# Autodesk Inventor assembly: AMR_assembly
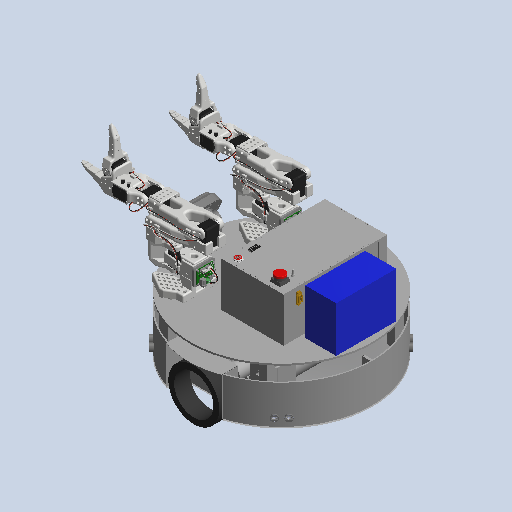
[picture p0: Inventor's stored thumbnail of the model, 512x512]
Saved by Autodesk Inventor 2026 (Build 300175050, 175E)
## iProperties
Part Number: AMR_assembly
Document SubType Name: Assembly
Designer: Kartik
Mass: 9467.85 g
Surface Area: 27408.7 cm^2
Volume: 7326.52 cm^3
Density: 1.29227 g/cm^3
Author: Kartik
## Documents named in this file (23)
- D:\Kartik\Projects\AMR\CAD\1 Assembly\AMR_assembly.iam
- D:\Kartik\Projects\AMR\CAD\3 Parts\AMR_base.ipt
- D:\Kartik\Projects\AMR\CAD\3 Parts\Wheel_Cover.ipt
- D:\Kartik\Projects\AMR\CAD\3 Parts\Wheel_rubber.ipt
- D:\Kartik\Projects\AMR\CAD\3 Parts\Motor.ipt
- D:\Kartik\Projects\AMR\CAD\3 Parts\Motor_mount.ipt
- D:\Kartik\Projects\AMR\CAD\3 Parts\Encoder.ipt
- D:\Kartik\Projects\AMR\CAD\2 Sub-assembly\PCB enclosure.iam
- D:\Kartik\Projects\AMR\CAD\6 Exports\STEP\SO101\SO101 Assembly\SO101 Assembly\SO101 Assembly.iam
- D:\Kartik\Projects\AMR\CAD\3 Parts\Pulley.ipt
- D:\Kartik\Projects\AMR\CAD\3 Parts\Frame_member.ipt
- D:\Kartik\Projects\AMR\CAD\3 Parts\LIdar_p2.ipt
- D:\Kartik\Projects\AMR\CAD\3 Parts\LIdar_p1.ipt
- D:\Kartik\Projects\AMR\CAD\3 Parts\layer2.ipt
- D:\Kartik\Projects\AMR\CAD\3 Parts\Battery.ipt
- D:\Kartik\Projects\AMR\CAD\4 Boughtouts\intel-realsense-depth-camera-d455\INTEL REALSENSE  DEPTH CAMERA D455\INTEL REALSENSE  DEPTH CAMERA D455\INTEL REALSENSE  DEPTH CAMERA D455\INTEL REALSENSE  DEPTH CAMERA D.ipt
- D:\Kartik\Projects\AMR\CAD\4 Boughtouts\intel-realsense-d455-mount-1\Assem1\Assem1\Assem1.ipt
- D:\Kartik\Projects\AMR\CAD\4 Boughtouts\hc-sr04-ultrasonic-sensor-12\Ultrasonic sensor\Ultrasonic sensor\Ultrasonic sensor.ipt
- D:\Kartik\Projects\AMR\CAD\3 Parts\Bottom_Enclosure_1.ipt
- D:\Kartik\Projects\AMR\CAD\3 Parts\Bottom_Enclosure_2.ipt
- D:\Kartik\Projects\AMR\CAD\2 Sub-assembly\PCB enclosure_v2.iam
- D:\Kartik\Projects\AMR\CAD\4 Boughtouts\emergency-stop-switch-1\Emergency stop switch\Emergency stop switch\Emergency stop switch.ipt
- D:\Kartik\Projects\AMR\CAD\4 Boughtouts\mini-toggle-switches-1\6mm SPDT Mini Toggle Switch\6mm SPDT Mini Toggle Switch\6mm SPDT Mini Toggle Switch.ipt
## Components (39 placed, 22 different names)
1. AMR_base:1 — Mate:1, Mate:2, Mate:3, Mate:4, Flush:1, Mate:6, Mate:8, Mate:25, Mate:27, Mate:28, Mate:29, Mate:30, Mate:31, Mate:32, Mate:33, Mate:34, Mate:39, Mate:55, Mate:56, Mate:57, Mate:58, Mate:59, Mate:60, Mate:61, Mate:62
2. Wheel_Cover:1 — Mate:1, Mate:2, Mate:3, Flush:2, Mate:10, Mate:23
3. Wheel_Cover:2 — Mate:4, Flush:1, Flush:2, Mate:9, Mate:24
4. Motor:1 — Flush:5, Mate:7, Flush:6, Mate:18, Mate:26
5. Motor:2 — Flush:3, Mate:5, Flush:4, Mate:16, Mate:25, Mate:26
6. Motor_mount:1 — Flush:5, Mate:7, Flush:6, Mate:8, Mate:17, Mate:24
7. Motor_mount:2 — Flush:3, Mate:5, Flush:4, Mate:6, Mate:15, Mate:23
8. Encoder:1 — Mate:12, Mate:19, Mate:20
9. Encoder:2 — Mate:13, Mate:21, Mate:22
10. Wheel_rubber:2 — Mate:10, Mate:11, Mate:12
11. Wheel_rubber:3 — Mate:9, Mate:11, Mate:13
12. PCB enclosure:1 [sub-assembly] — Mate:40
13. SO101 Assembly:1 [sub-assembly] — Mate:43, Flush:16, Mate:45, Flush:17
14. SO101 Assembly:2 [sub-assembly] — Mate:44, Flush:16, Mate:45, Flush:17
15. Pulley:1 — Mate:15, Mate:16
16. Pulley:2 — Mate:17, Mate:18
17. Pulley:3 — Mate:19, Mate:20
18. Pulley:4 — Mate:21, Mate:22
19. Frame_member:1 — Mate:27, Mate:28, Flush:14, Flush:15
20. Frame_member:2 — Mate:29, Mate:34, Flush:13
21. Frame_member:3 — Mate:30, Mate:33, Flush:13, Flush:14
22. Frame_member:4 — Mate:31, Mate:32, Flush:15
23. LIdar_p2:1 — Mate:36, Mate:37
24. LIdar_p1:1 — Mate:36, Mate:37, Mate:38
25. layer2:1 — Mate:39, Mate:40, Mate:43, Mate:44, Mate:49, Mate:38, Mate:75, Mate:76
26. Battery:1 — Mate:76, Mate:77
27. INTEL REALSENSE  DEPTH CAMERA D:1 — Mate:50, Mate:51, Mate:52
28. Assem1:1 — Mate:49, Mate:50, Mate:51, Mate:52
29. Ultrasonic sensor:1 — Mate:73, Mate:74
30. Ultrasonic sensor:2 — Mate:68, Mate:69
31. Ultrasonic sensor:3 — Mate:66, Mate:67
32. Ultrasonic sensor:4 — Mate:71, Mate:72
33. Bottom_Enclosure_1:1 — Mate:55, Mate:56, Mate:68, Mate:69
34. Bottom_Enclosure_1:2 — Mate:57, Mate:58, Mate:66, Mate:67, Mate:70
35. Bottom_Enclosure_2:1 — Mate:59, Mate:60, Mate:73, Mate:74
36. Bottom_Enclosure_2:2 — Mate:61, Mate:62, Mate:70, Mate:71, Mate:72
37. PCB enclosure_v2:1 [sub-assembly] — Mate:75, Mate:77, Mate:78, Mate:79
38. Emergency stop switch:1 — Mate:78
39. 6mm SPDT Mini Toggle Switch:1 — Mate:79
## Relationships (78: Mate 67, Flush 11)
- Mate:1: AMR_base:1 ↔ Wheel_Cover:1
- Mate:2: AMR_base:1 ↔ Wheel_Cover:1
- Mate:3: AMR_base:1 ↔ Wheel_Cover:1
- Mate:4: AMR_base:1 ↔ Wheel_Cover:2
- Flush:1: AMR_base:1 ↔ Wheel_Cover:2
- Flush:2: Wheel_Cover:1 ↔ Wheel_Cover:2
- Flush:3: Motor:2 ↔ Motor_mount:2
- Mate:5: Motor:2 ↔ Motor_mount:2
- Flush:4: Motor:2 ↔ Motor_mount:2
- Mate:6: AMR_base:1 ↔ Motor_mount:2
- Flush:5: Motor:1 ↔ Motor_mount:1
- Mate:7: Motor:1 ↔ Motor_mount:1
- Flush:6: Motor:1 ↔ Motor_mount:1
- Mate:8: AMR_base:1 ↔ Motor_mount:1
- Mate:9 (2 mm): Wheel_Cover:2 ↔ Wheel_rubber:3
- Mate:10 (2 mm): Wheel_Cover:1 ↔ Wheel_rubber:2
- Mate:11: Wheel_rubber:2 ↔ Wheel_rubber:3
- Mate:12: Encoder:1 ↔ Wheel_rubber:2
- Mate:13: Encoder:2 ↔ Wheel_rubber:3
- Mate:15: Motor_mount:2 ↔ Pulley:1
- Mate:16: Motor:2 ↔ Pulley:1
- Mate:17: Motor_mount:1 ↔ Pulley:2
- Mate:18: Motor:1 ↔ Pulley:2
- Mate:19: Encoder:1 ↔ Pulley:3
- Mate:20: Encoder:1 ↔ Pulley:3
- Mate:21: Encoder:2 ↔ Pulley:4
- Mate:22: Encoder:2 ↔ Pulley:4
- Mate:23 (62 mm): Wheel_Cover:1 ↔ Motor_mount:2
- Mate:24 (62 mm): Wheel_Cover:2 ↔ Motor_mount:1
- Mate:25 (-64 mm): AMR_base:1 ↔ Motor:2
- Mate:26 (128 mm): Motor:1 ↔ Motor:2
- Mate:27: AMR_base:1 ↔ Frame_member:1
- Mate:28: AMR_base:1 ↔ Frame_member:1
- Mate:29: AMR_base:1 ↔ Frame_member:2
- Mate:30: AMR_base:1 ↔ Frame_member:3
- Mate:31: AMR_base:1 ↔ Frame_member:4
- Mate:32: AMR_base:1 ↔ Frame_member:4
- Mate:33: AMR_base:1 ↔ Frame_member:3
- Mate:34: AMR_base:1 ↔ Frame_member:2
- Mate:36: LIdar_p2:1 ↔ LIdar_p1:1
- Mate:37: LIdar_p2:1 ↔ LIdar_p1:1
- Mate:38 (2 mm): LIdar_p1:1 ↔ layer2:1
- Flush:13: Frame_member:2 ↔ Frame_member:3
- Flush:14: Frame_member:1 ↔ Frame_member:3
- Flush:15: Frame_member:1 ↔ Frame_member:4
- Mate:39: AMR_base:1 ↔ layer2:1
- Mate:40: PCB enclosure:1 ↔ layer2:1
- Mate:43: SO101 Assembly:1 ↔ layer2:1
- Mate:44: SO101 Assembly:2 ↔ layer2:1
- Flush:16: SO101 Assembly:1 ↔ SO101 Assembly:2
- Mate:45 (100 mm): SO101 Assembly:1 ↔ SO101 Assembly:2
- Flush:17: SO101 Assembly:1 ↔ SO101 Assembly:2
- Mate:49: layer2:1 ↔ Assem1:1
- Mate:50: INTEL REALSENSE  DEPTH CAMERA D:1 ↔ Assem1:1
- Mate:51: INTEL REALSENSE  DEPTH CAMERA D:1 ↔ Assem1:1
- Mate:52: INTEL REALSENSE  DEPTH CAMERA D:1 ↔ Assem1:1
- Mate:55: AMR_base:1 ↔ Bottom_Enclosure_1:1
- Mate:56: AMR_base:1 ↔ Bottom_Enclosure_1:1
- Mate:57: AMR_base:1 ↔ Bottom_Enclosure_1:2
- Mate:58: AMR_base:1 ↔ Bottom_Enclosure_1:2
- Mate:59: AMR_base:1 ↔ Bottom_Enclosure_2:1
- Mate:60: AMR_base:1 ↔ Bottom_Enclosure_2:1
- Mate:61: AMR_base:1 ↔ Bottom_Enclosure_2:2
- Mate:62: AMR_base:1 ↔ Bottom_Enclosure_2:2
- Mate:66: Ultrasonic sensor:3 ↔ Bottom_Enclosure_1:2
- Mate:67: Ultrasonic sensor:3 ↔ Bottom_Enclosure_1:2
- Mate:68: Ultrasonic sensor:2 ↔ Bottom_Enclosure_1:1
- Mate:69: Ultrasonic sensor:2 ↔ Bottom_Enclosure_1:1
- Mate:70: Bottom_Enclosure_1:2 ↔ Bottom_Enclosure_2:2
- Mate:71: Ultrasonic sensor:4 ↔ Bottom_Enclosure_2:2
- Mate:72: Ultrasonic sensor:4 ↔ Bottom_Enclosure_2:2
- Mate:73: Ultrasonic sensor:1 ↔ Bottom_Enclosure_2:1
- Mate:74: Ultrasonic sensor:1 ↔ Bottom_Enclosure_2:1
- Mate:75 (10 mm): layer2:1 ↔ PCB enclosure_v2:1
- Mate:76: layer2:1 ↔ Battery:1
- Mate:77 (10 mm): Battery:1 ↔ PCB enclosure_v2:1
- Mate:78: PCB enclosure_v2:1 ↔ Emergency stop switch:1
- Mate:79: PCB enclosure_v2:1 ↔ 6mm SPDT Mini Toggle Switch:1
